# Autodesk Inventor assembly: Assembly
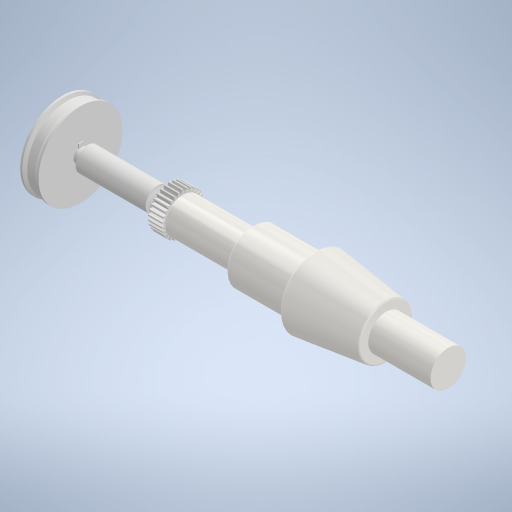
[picture p0: Inventor's stored thumbnail of the model, 512x512]
Saved by Autodesk Inventor 2024 (Build 280153000, 153)
## iProperties
Created: 2024-04-01
Part Number: Assembly
Document SubType Name: Assembly
Designer: rudyr
Author: rudyr
## Documents named in this file (7)
- C:\Users\rudyr\OneDrive\Desktop\URL\QUINTO CICLO\DINÁMICA LAB\Assembly.iam
- C:\Users\rudyr\Downloads\POLEA.ipt
- C:\Users\rudyr\Downloads\ENGRANE.ipt
- C:\Users\rudyr\Downloads\EJE_CUÑEROS.ipt
- C:\Users\rudyr\Downloads\CUÑA.ipt
- C:\Users\rudyr\OneDrive\Desktop\URL\QUINTO CICLO\DINÁMICA LAB\Compress Spring11.ipt
- C:\Users\rudyr\OneDrive\Desktop\URL\QUINTO CICLO\DINÁMICA LAB\Shaft1.ipt
## Components (7 placed, 6 different names)
1. POLEA:1 — Rigid:1, Slider:1
2. ENGRANE:1 — Rigid:2
3. CUÑA:1 — Rigid:4, Flush:2
4. CUÑA:2 — Rigid:3, Flush:1
5. EJE_CUÑEROS:1 — Rigid:1, Slider:1, Rigid:2, Rigid:3, Flush:1, Rigid:4, Flush:2, Mate:1
6. Compress Spring1:1
7. Shaft:1 — Mate:1
## Relationships (8: WeldJoint 4, Flush 2, TranslationJoint 1, Mate 1)
- Rigid:1 [WeldJoint]: POLEA:1 ↔ EJE_CUÑEROS:1
- Slider:1 [TranslationJoint]: POLEA:1 ↔ EJE_CUÑEROS:1
- Rigid:2 [WeldJoint]: ENGRANE:1 ↔ EJE_CUÑEROS:1
- Rigid:3 [WeldJoint]: CUÑA:2 ↔ EJE_CUÑEROS:1
- Flush:1: CUÑA:2 ↔ EJE_CUÑEROS:1
- Rigid:4 [WeldJoint]: CUÑA:1 ↔ EJE_CUÑEROS:1
- Flush:2: CUÑA:1 ↔ EJE_CUÑEROS:1
- Mate:1: EJE_CUÑEROS:1 ↔ Shaft:1
